# Autodesk Inventor assembly: PushrodLeftNCS
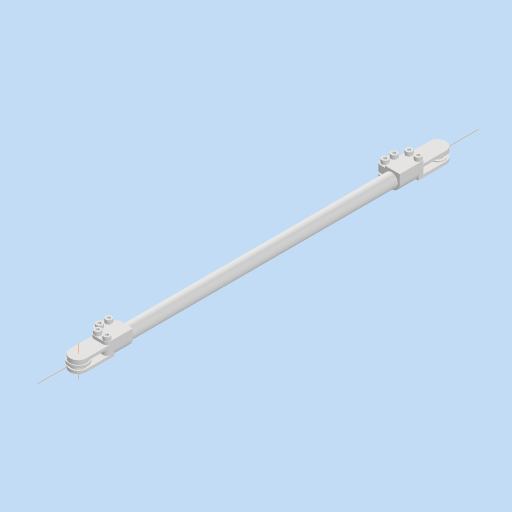
[picture p0: Inventor's stored thumbnail of the model, 512x512]
Saved by Autodesk Inventor 2023 (Build 270158000, 158)
## iProperties
Created: 2026-06-18
Part Number: PushrodLeftNCS
Document SubType Name: Assembly
Designer: Nathann
Author: Nathann
## Documents named in this file (2)
- C:\Users\Nathann\ClawdDrive\Objet3D\RunningRobot\PartURDF\PushrodLeftNCS.iam
- C:\Users\Nathann\ClawdDrive\Objet3D\RunningRobot\PartURDF\PushrodLeft.iam
## Components (1 placed, 1 different names)
1. PushrodLeft:1 [sub-assembly] — Mate:1, Mate:2, Mate:5, Mate:6
## Relationships (6: Mate 6)
- Mate:1: PushrodLeft:1
- Mate:2: PushrodLeft:1
- Mate:3
- Mate:4
- Mate:5: PushrodLeft:1
- Mate:6: PushrodLeft:1
